# Autodesk Inventor assembly: Ensamble TensionCompresion
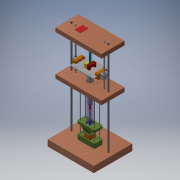
[picture p0: Inventor's stored thumbnail of the model, 180x180]
Saved by Autodesk Inventor 2018 (Build 220112000, 112)
## iProperties
Created: 2019-05-18
Part Number: Ensamble TensionCompresion
Document SubType Name: Assembly
Designer: JLVega003
Author: JLVega003
## Documents named in this file (31)
- C:\Users\Ivan\Documents\GitHub\RMTestMachine\3DModel\Ensamble TensionCompresion.iam
- C:\Users\Ivan\Documents\GitHub\RMTestMachine\3DModel\sujetador motor.ipt
- C:\Users\Ivan\Documents\GitHub\RMTestMachine\3DModel\motor con reductora.ipt
- C:\Users\Ivan\Documents\GitHub\RMTestMachine\3DModel\acople.ipt
- C:\Users\Ivan\Documents\GitHub\RMTestMachine\3DModel\sujetador motor guia.ipt
- C:\Users\Ivan\Documents\GitHub\RMTestMachine\3DModel\sujetador guia ejercedor presion.ipt
- C:\Users\Ivan\Documents\GitHub\RMTestMachine\3DModel\barra t8.ipt
- C:\Users\Ivan\Documents\GitHub\RMTestMachine\3DModel\barra solida hueca.ipt
- C:\Users\Ivan\Documents\GitHub\RMTestMachine\3DModel\tuerca anti backlash.ipt
- C:\Users\Ivan\Documents\GitHub\RMTestMachine\3DModel\base inferior.ipt
- C:\Users\Ivan\Documents\GitHub\RMTestMachine\3DModel\sujetador plancha aluminio.ipt
- C:\Users\Ivan\Documents\GitHub\RMTestMachine\3DModel\cojinete lineal.ipt
- C:\Users\Ivan\Documents\GitHub\RMTestMachine\3DModel\barra lisa 8mm.ipt
- C:\Users\Ivan\Documents\GitHub\RMTestMachine\3DModel\sujetador plancha aluminio_MIR1.ipt
- C:\Users\Ivan\Documents\GitHub\RMTestMachine\3DModel\cojinete lineal_MIR.ipt
- C:\Users\Ivan\Documents\GitHub\RMTestMachine\3DModel\barra lisa 8mm_MIR.ipt
- C:\Users\Ivan\Documents\GitHub\RMTestMachine\3DModel\sujetador inferior.ipt
- C:\Users\Ivan\Documents\GitHub\RMTestMachine\3DModel\sujetador movil.ipt
- C:\Users\Ivan\Documents\GitHub\RMTestMachine\3DModel\base de madera pequeña.ipt
- C:\Users\Ivan\Documents\GitHub\RMTestMachine\3DModel\base de madera pequeña - superior.ipt
- C:\Users\Ivan\Documents\GitHub\RMTestMachine\3DModel\barras M10.ipt
- C:\Users\Ivan\Documents\GitHub\RMTestMachine\3DModel\base superior.ipt
- C:\Users\Ivan\Documents\GitHub\RMTestMachine\3DModel\soportes celda de carga.ipt
- C:\Users\Ivan\Documents\GitHub\RMTestMachine\3DModel\celda de carga.ipt
- C:\Users\Ivan\Documents\GitHub\RMTestMachine\3DModel\soportes celda de carga - m4.ipt
- C:\Users\Ivan\Documents\GitHub\RMTestMachine\3DModel\barra espaciadora.ipt
- C:\Users\Ivan\Documents\GitHub\RMTestMachine\3DModel\base de madera grande.ipt
- C:\Users\Ivan\Documents\GitHub\RMTestMachine\3DModel\Pieza Prueba.ipt
- C:\Users\Ivan\Documents\GitHub\RMTestMachine\3DModel\barras M4.ipt
- C:\Users\Ivan\Documents\GitHub\RMTestMachine\3DModel\barras M4 medium.ipt
- C:\Users\Ivan\Documents\GitHub\RMTestMachine\3DModel\barras M4 small.ipt
## Components (43 placed, 30 different names)
1. sujetador motor:1 — Flush:1, Flush:2, Mate:1, Mate:2, Mate:3, Mate:8, Flush:3, Insert:21, Mate:38, Mate:48, Mate:49, Mate:50
2. motor con reductora:1 — Mate:1, Mate:2, Mate:3, Mate:4, Mate:5, Mate:6, Mate:7, Mate:9, Mate:12
3. acople:1 — Mate:4, Mate:5, Mate:11
4. sujetador motor guia:1 — Mate:6, Mate:7, Mate:8, Mate:10, Insert:20, Mate:44
5. sujetador guia ejercedor presion:1 — Mate:9, Mate:10, Insert:9, Insert:19, Mate:51, Mate:52, Mate:53
6. barra t8:1 — Mate:11, Mate:12, Mate:14
7. barra solida hueca:1 — Mate:13, Mate:14, Mate:15, Insert:2, Mate:25, Insert:23
8. tuerca anti backlash:1 — Mate:13, Insert:23
9. base inferior:1 — Mate:15, Insert:2, Flush:3, Insert:3, Mate:16, Insert:6, Mate:21, Insert:7, Mate:22
10. sujetador plancha aluminio:2 — Insert:3, Mate:16, Insert:4, Mate:17, Mate:37
11. cojinete lineal:1 — Insert:4, Mate:17, Mate:18
12. barra lisa 8mm:1 — Mate:18, Flush:4, Flush:6
13. sujetador plancha aluminio_MIR1:1 — Mate:19, Insert:5, Insert:6, Mate:21
14. cojinete lineal_MIR:1 — Mate:19, Insert:5, Mate:20
15. barra lisa 8mm_MIR:1 — Mate:20, Flush:4
16. sujetador inferior:1 — Insert:7, Mate:22, Insert:8, Mate:23
17. sujetador movil:1 — Insert:8, Mate:23, Mate:41
18. base de madera pequeña:1 — Insert:9, Mate:24, Mate:36, Mate:37, Flush:6, Mate:51, Mate:52, Insert:24, Insert:25, Insert:26, Insert:27, Mate:53
19. base de madera pequeña - superior:1 — Mate:25, Mate:26, Mate:27, Insert:11, Mate:28, Insert:12, Mate:29, Mate:36
20. barras M10:1 — Flush:5, Insert:22
21. barras M10:2 — Mate:27, Flush:5
22. base superior:1 — Insert:17, Mate:34, Insert:18, Mate:35
23. soportes celda de carga:1 — Insert:11, Mate:28, Insert:13, Mate:30
24. soportes celda de carga:2 — Insert:12, Mate:29
25. celda de carga:1 — Insert:13, Mate:30, Insert:14, Mate:31, Mate:34
26. soportes celda de carga - m4:1 — Insert:14, Mate:31, Insert:17
27. sujetador inferior:2 — Insert:18, Mate:35, Flush:7, Mate:39, Angle:1, Flush:8
28. sujetador movil:2 — Mate:40
29. barra espaciadora:1 — Insert:19, Insert:20
30. base de madera grande:1 — Insert:21, Mate:38, Insert:22, Mate:42, Mate:43, Mate:45, Mate:46, Mate:47, Insert:28, Insert:29, Insert:30, Insert:31
31. Pieza Prueba:1 — Flush:7, Mate:39, Angle:1, Flush:8, Mate:40, Mate:41
32. barras M4:1 — Mate:43, Mate:44
33. barras M4:2 — Mate:47, Mate:48
34. barras M4:3 — Mate:45, Mate:49
35. barras M4:4 — Mate:46, Mate:50
36. barras M4 small:1 — Insert:28
37. barras M4 medium:2 — Insert:24
38. barras M4 medium:3 — Insert:25
39. barras M4 medium:4 — Insert:26
40. barras M4 medium:5 — Insert:27
41. barras M4 small:2 — Insert:29
42. barras M4 small:3 — Insert:30
43. barras M4 small:4 — Insert:31
## Relationships (89: Mate 52, Insert 28, Flush 8, Angle 1)
- Flush:1: sujetador motor:1
- Flush:2: sujetador motor:1
- Mate:1: sujetador motor:1 ↔ motor con reductora:1
- Mate:2: sujetador motor:1 ↔ motor con reductora:1
- Mate:3: sujetador motor:1 ↔ motor con reductora:1
- Mate:4: motor con reductora:1 ↔ acople:1
- Mate:5 (3.5 mm): motor con reductora:1 ↔ acople:1
- Mate:6: motor con reductora:1 ↔ sujetador motor guia:1
- Mate:7: motor con reductora:1 ↔ sujetador motor guia:1
- Mate:8: sujetador motor:1 ↔ sujetador motor guia:1
- Mate:9: motor con reductora:1 ↔ sujetador guia ejercedor presion:1
- Mate:10: sujetador motor guia:1 ↔ sujetador guia ejercedor presion:1
- Mate:11: acople:1 ↔ barra t8:1
- Mate:12 (1 mm): motor con reductora:1 ↔ barra t8:1
- Mate:13: barra solida hueca:1 ↔ tuerca anti backlash:1
- Mate:14: barra t8:1 ↔ barra solida hueca:1
- Mate:15: barra solida hueca:1 ↔ base inferior:1
- Insert:2: barra solida hueca:1 ↔ base inferior:1
- Flush:3: sujetador motor:1 ↔ base inferior:1
- Insert:3: base inferior:1 ↔ sujetador plancha aluminio:2
- Mate:16: base inferior:1 ↔ sujetador plancha aluminio:2
- Insert:4: sujetador plancha aluminio:2 ↔ cojinete lineal:1
- Mate:17: sujetador plancha aluminio:2 ↔ cojinete lineal:1
- Mate:18: cojinete lineal:1 ↔ barra lisa 8mm:1
- Mate:19: sujetador plancha aluminio_MIR1:1 ↔ cojinete lineal_MIR:1
- Insert:5: sujetador plancha aluminio_MIR1:1 ↔ cojinete lineal_MIR:1
- Mate:20: cojinete lineal_MIR:1 ↔ barra lisa 8mm_MIR:1
- Insert:6: base inferior:1 ↔ sujetador plancha aluminio_MIR1:1
- Mate:21: base inferior:1 ↔ sujetador plancha aluminio_MIR1:1
- Flush:4: barra lisa 8mm:1 ↔ barra lisa 8mm_MIR:1
- Insert:7: base inferior:1 ↔ sujetador inferior:1
- Mate:22: base inferior:1 ↔ sujetador inferior:1
- Insert:8: sujetador inferior:1 ↔ sujetador movil:1
- Mate:23: sujetador inferior:1 ↔ sujetador movil:1
- Insert:9: sujetador guia ejercedor presion:1 ↔ base de madera pequeña:1
- Mate:24: base de madera pequeña:1
- Mate:25: barra solida hueca:1 ↔ base de madera pequeña - superior:1
- Mate:26: base de madera pequeña - superior:1
- Mate:27: base de madera pequeña - superior:1 ↔ barras M10:2
- Flush:5: barras M10:1 ↔ barras M10:2
- Insert:11: base de madera pequeña - superior:1 ↔ soportes celda de carga:1
- Mate:28: base de madera pequeña - superior:1 ↔ soportes celda de carga:1
- Insert:12: base de madera pequeña - superior:1 ↔ soportes celda de carga:2
- Mate:29: base de madera pequeña - superior:1 ↔ soportes celda de carga:2
- Insert:13: soportes celda de carga:1 ↔ celda de carga:1
- Mate:30: soportes celda de carga:1 ↔ celda de carga:1
- Insert:14: celda de carga:1 ↔ soportes celda de carga - m4:1
- Mate:31: celda de carga:1 ↔ soportes celda de carga - m4:1
- [Insert]: sujetador inferior:2 ↔ sujetador movil:2
- [Mate]: sujetador inferior:2 ↔ sujetador movil:2
- Insert:17: base superior:1 ↔ soportes celda de carga - m4:1
- Mate:34: base superior:1 ↔ celda de carga:1
- Insert:18: base superior:1 ↔ sujetador inferior:2
- Mate:35: base superior:1 ↔ sujetador inferior:2
- Insert:19: sujetador guia ejercedor presion:1 ↔ barra espaciadora:1
- Insert:20: sujetador motor guia:1 ↔ barra espaciadora:1
- Mate:36 (237 mm): base de madera pequeña:1 ↔ base de madera pequeña - superior:1
- Mate:37: sujetador plancha aluminio:2 ↔ base de madera pequeña:1
- Flush:6 (-10 mm): barra lisa 8mm:1 ↔ base de madera pequeña:1
- Insert:21: sujetador motor:1 ↔ base de madera grande:1
- Mate:38: sujetador motor:1 ↔ base de madera grande:1
- Insert:22: barras M10:1 ↔ base de madera grande:1
- Flush:7: sujetador inferior:2 ↔ Pieza Prueba:1
- Mate:39: sujetador inferior:2 ↔ Pieza Prueba:1
- Angle:1 (0 deg): sujetador inferior:2 ↔ Pieza Prueba:1
- Flush:8 (-16.5 mm): sujetador inferior:2 ↔ Pieza Prueba:1
- Mate:40: sujetador movil:2 ↔ Pieza Prueba:1
- Mate:41: sujetador movil:1 ↔ Pieza Prueba:1
- Mate:42: base de madera grande:1
- Insert:23: barra solida hueca:1 ↔ tuerca anti backlash:1
- Mate:43: base de madera grande:1 ↔ barras M4:1
- Mate:44: sujetador motor guia:1 ↔ barras M4:1
- Mate:45: base de madera grande:1 ↔ barras M4:3
- Mate:46: base de madera grande:1 ↔ barras M4:4
- Mate:47: base de madera grande:1 ↔ barras M4:2
- Mate:48: sujetador motor:1 ↔ barras M4:2
- Mate:49: sujetador motor:1 ↔ barras M4:3
- Mate:50: sujetador motor:1 ↔ barras M4:4
- Mate:51: sujetador guia ejercedor presion:1 ↔ base de madera pequeña:1
- Mate:52: sujetador guia ejercedor presion:1 ↔ base de madera pequeña:1
- Insert:24 (-5 mm): base de madera pequeña:1 ↔ barras M4 medium:2
- Insert:25 (-5 mm): base de madera pequeña:1 ↔ barras M4 medium:3
- Insert:26 (5 mm): base de madera pequeña:1 ↔ barras M4 medium:4
- Insert:27 (5 mm): base de madera pequeña:1 ↔ barras M4 medium:5
- Insert:28: base de madera grande:1 ↔ barras M4 small:1
- Insert:29: base de madera grande:1 ↔ barras M4 small:2
- Insert:30: base de madera grande:1 ↔ barras M4 small:3
- Insert:31: base de madera grande:1 ↔ barras M4 small:4
- Mate:53: sujetador guia ejercedor presion:1 ↔ base de madera pequeña:1
## Named parameters: d55_d34 = 0 mm, d56_d35 = 30 mm, d57_d36 = 0 mm, d58_d33 = 0 mm
